# Autodesk Inventor assembly: 200-00
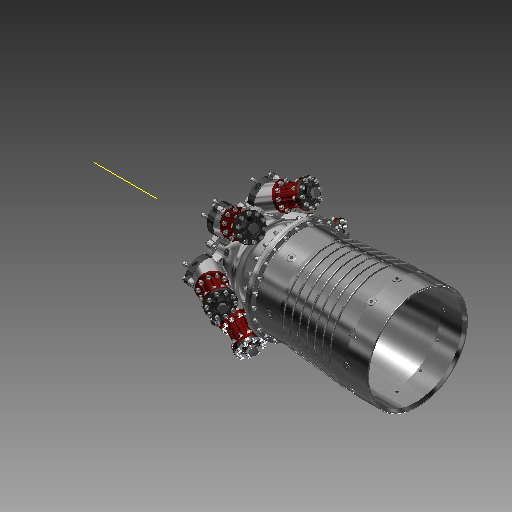
[picture p0: Inventor's stored thumbnail of the model, 512x512]
Saved by Autodesk Inventor 2019 (Build 230136000, 136)
## iProperties
Company: Autodesk Inc.
Created: 2017-03-14
Part Number: 200-00
Document SubType Name: Assembly
Designer: Autodesk Inc.
Mass: 14006.2 g
Surface Area: 11561.7 cm^2
Volume: 2946.17 cm^3
Density: 4.75401 g/cm^3
Author: Inventor
## Documents named in this file (9)
- C:\TEMP\Jet Engine Model\Workspace\Combustion Stage.iam
- C:\TEMP\Jet Engine Model\Workspace\Front Compression Fan\Combustion Shell.ipt
- C:\TEMP\Jet Engine Model\Workspace\Front Compression Fan\Combustion Chamber.iam
- C:\TEMP\Jet Engine Model\Workspace\Front Compression Fan\Intake Casing.ipt
- C:\TEMP\Jet Engine Model\Workspace\Design Accelerator\Bolted Connection1.iam
- C:\TEMP\Jet Engine Model\Workspace\Front Compression Fan\Combustion C-Ring.ipt
- C:\TEMP\Jet Engine Model\Libraries\Content Center Files\en-US\ISO 10642(1)\ISO 10642 - M6 x  25.ipt
- C:\TEMP\Jet Engine Model\Libraries\Content Center Files\en-US\ISO 4762(2)\ISO 4762 - M5 x 20ISO.ipt
- C:\TEMP\Jet Engine Model\Libraries\Content Center Files\en-US\ISO 4762(2)\ISO 4762 - M5 x 16ISO.ipt
## Components (138 placed, 8 different names)
1. Combustion Shell:1 — Mate:4, Insert:4, Insert:9, Flush:6, Flush:7, Flush:8, Mate:5, Mate:6, Mate:7, Mate:10, Mate:12, Mate:13, Mate:14
2. Intake Casing:1 — Mate:5, Mate:6, Mate:7, Mate:8, Mate:9
3. Combustion Chamber:1 [sub-assembly] — Mate:10
4. Combustion Chamber:2 [sub-assembly]
5. Combustion Chamber:3 [sub-assembly]
6. Combustion Chamber:4 [sub-assembly] — Insert:8
7. Combustion Chamber:5 [sub-assembly]
8. Combustion Chamber:6 [sub-assembly]
9. ISO 10642 M6 x  25:4 — Insert:4
10. ISO 10642 M6 x  25:5
11. ISO 10642 M6 x  25:6
12. ISO 4762 M5 x 20:49 — Insert:5
13. ISO 4762 M5 x 20:55 — Insert:6
14. ISO 4762 M5 x 20:50
15. ISO 4762 M5 x 20:56
16. ISO 4762 M5 x 20:51
17. ISO 4762 M5 x 20:57
18. ISO 4762 M5 x 20:52
19. ISO 4762 M5 x 20:58
20. ISO 4762 M5 x 20:53
21. ISO 4762 M5 x 20:59
22. ISO 4762 M5 x 20:54
23. ISO 4762 M5 x 20:60
24. ISO 4762 M5 x 16:67 — Insert:7
25. ISO 4762 M5 x 16:68
26. ISO 4762 M5 x 16:69
27. ISO 4762 M5 x 16:70
28. ISO 4762 M5 x 16:71
29. ISO 4762 M5 x 16:72
30. ISO 4762 M5 x 20:61 — Insert:9
31. ISO 4762 M5 x 20:62
32. ISO 4762 M5 x 20:63
33. ISO 4762 M5 x 20:64
34. ISO 4762 M5 x 20:65
35. ISO 4762 M5 x 20:66
36. ISO 4762 M5 x 20:67 — Insert:10
37. ISO 4762 M5 x 20:73 — Insert:11
38. ISO 4762 M5 x 20:68
39. ISO 4762 M5 x 20:74
40. ISO 4762 M5 x 20:69
41. ISO 4762 M5 x 20:75
42. ISO 4762 M5 x 20:70
43. ISO 4762 M5 x 20:76
44. ISO 4762 M5 x 20:71
45. ISO 4762 M5 x 20:77
46. ISO 4762 M5 x 20:72
47. ISO 4762 M5 x 20:78
48. Bolted Connection:1 [sub-assembly] — Mate:8, Mate:9
49. Bolted Connection:2 [sub-assembly]
50. Bolted Connection:3 [sub-assembly]
51. Bolted Connection:4 [sub-assembly]
52. Bolted Connection:5 [sub-assembly]
53. Bolted Connection:6 [sub-assembly]
54. Bolted Connection:7 [sub-assembly]
55. Bolted Connection:8 [sub-assembly]
56. Bolted Connection:9 [sub-assembly]
57. Bolted Connection:10 [sub-assembly]
58. Bolted Connection:11 [sub-assembly]
59. Bolted Connection:12 [sub-assembly]
60. Bolted Connection:13 [sub-assembly]
61. Bolted Connection:14 [sub-assembly]
62. Bolted Connection:15 [sub-assembly]
63. Bolted Connection:16 [sub-assembly]
64. Bolted Connection:17 [sub-assembly]
65. Bolted Connection:18 [sub-assembly]
66. Bolted Connection:19 [sub-assembly]
67. Bolted Connection:20 [sub-assembly]
68. Bolted Connection:21 [sub-assembly]
69. Bolted Connection:22 [sub-assembly]
70. Bolted Connection:23 [sub-assembly]
71. Bolted Connection:24 [sub-assembly]
72. Bolted Connection:25 [sub-assembly]
73. Combustion C-Ring:1 — Insert:5, Insert:6, Insert:7, Insert:10, Insert:11, Mate:12, Mate:13, Mate:14
74. Combustion C-Ring:2
75. Combustion C-Ring:3
76. Combustion C-Ring:4
77. Combustion C-Ring:5
78. Combustion C-Ring:6
79. ISO 4762 M5 x 16:2 — Insert:8
80. ISO 4762 M5 x 16:3
81. ISO 4762 M5 x 16:4
82. ISO 4762 M5 x 16:5
83. ISO 4762 M5 x 16:6
84. ISO 4762 M5 x 16:7
85. ISO 4762 M5 x 16:8
86. ISO 4762 M5 x 16:9
87. ISO 4762 M5 x 16:10
88. ISO 4762 M5 x 16:11
89. ISO 4762 M5 x 16:13
90. ISO 4762 M5 x 16:14
91. ISO 4762 M5 x 16:15
92. ISO 4762 M5 x 16:16
93. ISO 4762 M5 x 16:17
94. ISO 4762 M5 x 16:18
95. ISO 4762 M5 x 16:19
96. ISO 4762 M5 x 16:20
97. ISO 4762 M5 x 16:21
98. ISO 4762 M5 x 16:22
99. ISO 4762 M5 x 16:24
100. ISO 4762 M5 x 16:25
101. ISO 4762 M5 x 16:26
102. ISO 4762 M5 x 16:27
103. ISO 4762 M5 x 16:28
104. ISO 4762 M5 x 16:29
105. ISO 4762 M5 x 16:30
106. ISO 4762 M5 x 16:31
107. ISO 4762 M5 x 16:32
108. ISO 4762 M5 x 16:33
109. ISO 4762 M5 x 16:35
110. ISO 4762 M5 x 16:36
111. ISO 4762 M5 x 16:37
112. ISO 4762 M5 x 16:38
113. ISO 4762 M5 x 16:39
114. ISO 4762 M5 x 16:40
115. ISO 4762 M5 x 16:41
116. ISO 4762 M5 x 16:42
117. ISO 4762 M5 x 16:43
118. ISO 4762 M5 x 16:44
119. ISO 4762 M5 x 16:46
120. ISO 4762 M5 x 16:47
121. ISO 4762 M5 x 16:48
122. ISO 4762 M5 x 16:49
123. ISO 4762 M5 x 16:50
124. ISO 4762 M5 x 16:51
125. ISO 4762 M5 x 16:52
126. ISO 4762 M5 x 16:53
127. ISO 4762 M5 x 16:54
128. ISO 4762 M5 x 16:55
129. ISO 4762 M5 x 16:57
130. ISO 4762 M5 x 16:58
131. ISO 4762 M5 x 16:59
132. ISO 4762 M5 x 16:60
133. ISO 4762 M5 x 16:61
134. ISO 4762 M5 x 16:62
135. ISO 4762 M5 x 16:63
136. ISO 4762 M5 x 16:64
137. ISO 4762 M5 x 16:65
138. ISO 4762 M5 x 16:66
## Component patterns: (6 elements, first: Combustion Chamber:1), (3 elements, first: ISO 10642 M6 x  25:4), (6 elements, first: ISO 4762 M5 x 20:49 + ISO 4762 M5 x 20:55), (6 elements, first: ISO 4762 M5 x 16:67), (6 elements, first: ISO 4762 M5 x 20:61), (6 elements, first: ISO 4762 M5 x 20:67 + ISO 4762 M5 x 20:73), (25 elements, first: Bolted Connection:1), (6 elements, first: Combustion C-Ring:1), (10 elements, first: ISO 4762 M5 x 16:2), Component Pattern 4:2 (10 elements), Component Pattern 4:3 (10 elements), Component Pattern 4:4 (10 elements), Component Pattern 4:5 (10 elements), Component Pattern 4:6 (10 elements)
## Relationships (23: Mate 11, Insert 8, Flush 4)
- [Mate]: Combustion Shell:1 ↔ Combustion Chamber:1
- [Flush]: Combustion Shell:1 ↔ Combustion Chamber:1
- Mate:4: Combustion Shell:1
- Insert:4: Combustion Shell:1 ↔ ISO 10642 M6 x  25:4
- Insert:5: ISO 4762 M5 x 20:49 ↔ Combustion C-Ring:1
- Insert:6: ISO 4762 M5 x 20:55 ↔ Combustion C-Ring:1
- Insert:7: ISO 4762 M5 x 16:67 ↔ Combustion C-Ring:1
- Insert:8: Combustion Chamber:4 ↔ ISO 4762 M5 x 16:2
- Insert:9: Combustion Shell:1 ↔ ISO 4762 M5 x 20:61
- Insert:10 (11 mm): ISO 4762 M5 x 20:67 ↔ Combustion C-Ring:1
- Insert:11 (11 mm): ISO 4762 M5 x 20:73 ↔ Combustion C-Ring:1
- Flush:6: Combustion Shell:1
- Flush:7: Combustion Shell:1
- Flush:8: Combustion Shell:1
- Mate:5: Combustion Shell:1 ↔ Intake Casing:1
- Mate:6: Combustion Shell:1 ↔ Intake Casing:1
- Mate:7: Combustion Shell:1 ↔ Intake Casing:1
- Mate:8: Intake Casing:1 ↔ Bolted Connection:1
- Mate:9: Intake Casing:1 ↔ Bolted Connection:1
- Mate:10: Combustion Shell:1 ↔ Combustion Chamber:1
- Mate:12: Combustion Shell:1 ↔ Combustion C-Ring:1
- Mate:13: Combustion Shell:1 ↔ Combustion C-Ring:1
- Mate:14: Combustion Shell:1 ↔ Combustion C-Ring:1
